# Autodesk Inventor assembly: Dummy_radio_w_case
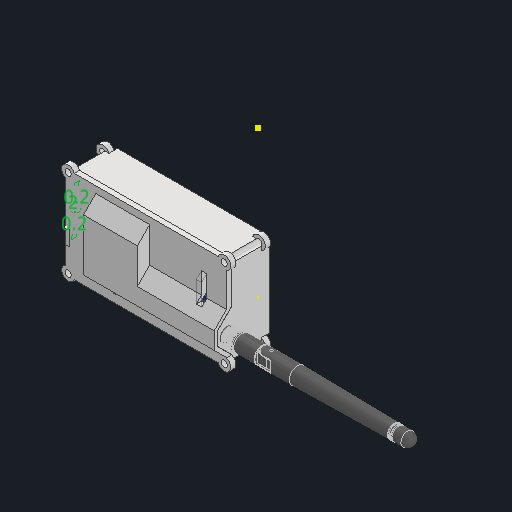
[picture p0: Inventor's stored thumbnail of the model, 512x512]
Saved by Autodesk Inventor 2026.2 (Build 302298000, 298)
## iProperties
Created: 2026-04-11
Part Number: Dummy_radio_w_case
Document SubType Name: Assembly
Designer: Malthe Sennels
Author: Malthe Sennels
## Documents named in this file (7)
- C:\Users\Malthe Sennels\OneDrive - Aalborg Universitet\ESD 610 - General\Inventor\Dummy_Radio\Dummy_radio_w_case.iam
- C:\Users\Malthe Sennels\OneDrive - Aalborg Universitet\ESD 610 - General\Inventor\Dummy_Radio\PCB.ipt
- C:\Users\Malthe Sennels\OneDrive - Aalborg Universitet\ESD 610 - General\Inventor\Dummy_Radio\GPS.ipt
- C:\Users\Malthe Sennels\OneDrive - Aalborg Universitet\ESD 610 - General\Inventor\Dummy_Radio\NRF24.ipt
- C:\Users\Malthe Sennels\OneDrive - Aalborg Universitet\ESD 610 - General\Inventor\Dummy_Radio\Buttom_case.ipt
- C:\Users\Malthe Sennels\OneDrive - Aalborg Universitet\ESD 610 - General\Inventor\Dummy_Radio\Top_case.ipt
- C:\Users\Malthe Sennels\OneDrive - Aalborg Universitet\ESD 610 - General\Inventor\Dummy_Radio\Light_guide.ipt
## Components (6 placed, 6 different names)
1. PCB:1 — Mate:1, Mate:2, Flush:1, Flush:2, Flush:3, Mate:3, Flush:4
2. GPS:1 — Mate:1, Mate:2, Flush:1
3. NRF24:1 — Flush:2, Flush:3, Mate:3
4. Buttom_case:1 — Flush:4, Flush:5
5. Top_case:1 — Flush:5, Flush:6
6. Light_guide:1 — Flush:6
## Relationships (9: Flush 6, Mate 3)
- Mate:1 (1 mm): PCB:1 ↔ GPS:1
- Mate:2 (1 mm): PCB:1 ↔ GPS:1
- Flush:1: PCB:1 ↔ GPS:1
- Flush:2: PCB:1 ↔ NRF24:1
- Flush:3: PCB:1 ↔ NRF24:1
- Mate:3: PCB:1 ↔ NRF24:1
- Flush:4: PCB:1 ↔ Buttom_case:1
- Flush:5: Buttom_case:1 ↔ Top_case:1
- Flush:6: Top_case:1 ↔ Light_guide:1
